# Autodesk Inventor assembly: Assembly1
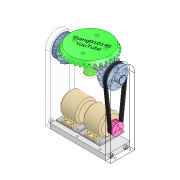
[picture p0: Inventor's stored thumbnail of the model, 180x180]
Saved by Autodesk Inventor 2022.5 (Build 265521000, 521)
## iProperties
Created: 2020-07-24
Part Number: Assembly1
Document SubType Name: Assembly
Designer: admin
Author: admin
## Documents named in this file (12)
- F:\YouTube\2024\YouTube\11N\6BevelGear2DoF\Assembly0.iam
- F:\YouTube\2024\YouTube\11N\6BevelGear2DoF\B32x2i2.ipt
- F:\YouTube\2024\YouTube\11N\6BevelGear2DoF\B16x2i2.ipt
- F:\YouTube\2024\YouTube\11N\6BevelGear2DoF\Cross.ipt
- F:\YouTube\2024\YouTube\11N\6BevelGear2DoF\Bearing.ipt
- F:\YouTube\2024\YouTube\11N\6BevelGear2DoF\Bottom.ipt
- F:\YouTube\2024\YouTube\11N\6BevelGear2DoF\Motor1x40.ipt
- F:\YouTube\2024\YouTube\11N\6BevelGear2DoF\Pulley.ipt
- F:\YouTube\2024\YouTube\11N\6BevelGear2DoF\Belt.ipt
- F:\YouTube\2024\YouTube\11N\6BevelGear2DoF\MotorBase.ipt
- F:\YouTube\2024\YouTube\11N\6BevelGear2DoF\PinScrew.ipt
- F:\YouTube\2024\YouTube\11N\6BevelGear2DoF\Nut3.ipt
## Components (16 placed, 11 different names)
1. Motor1x40:1 — Mate:18, Mate:19, Flush:4, Mate:22, Mate:23, Mate:25, Mate:31, Flush:6
2. Motor1x40:2 — Mate:21, Flush:4, Mate:32
3. Bearing:1 — Mate:12, Mate:13, Angle:1, Flush:1, Mate:18, Mate:24, Mate:26, Mate:27, Mate:28
4. Bearing:2 — Mate:14, Mate:15, Flush:1, Flush:2, Flush:3, Mate:16, Mate:21, Mate:33
5. Bottom:1 — Flush:2, Flush:3, Mate:16, Flush:5
6. Belt:1 — Mate:24, Mate:25, Mate:26
7. MotorBase:1 — Mate:31, Flush:5, Flush:6, Flush:7
8. MotorBase:2 — Mate:32, Flush:7, Mate:33, Insert:1, Insert:2, Insert:3
9. PinScrew:1 — Insert:1
10. Nut3:1 — Insert:2
11. Nut3:2 — Insert:3
12. B32x2i2:1 — Mate:29, Mate:30, Angle:2
13. B16x2i2:1 — Mate:3, Mate:4, Mate:5, Mate:7, Mate:12, Mate:13
14. B16x2i2:2 — Mate:6, Mate:7, Mate:14, Mate:15
15. Cross:1 — Mate:27, Mate:28, Mate:29, Mate:30
16. Pulley:1 — Mate:22, Mate:23
## Relationships (37: Mate 25, Flush 7, Insert 3, Angle 2)
- Mate:3: B16x2i2:1
- Mate:4: B16x2i2:1
- Mate:5: B16x2i2:1
- Mate:6: B16x2i2:2
- Mate:7: B16x2i2:1 ↔ B16x2i2:2
- Mate:12: Bearing:1 ↔ B16x2i2:1
- Mate:13: Bearing:1 ↔ B16x2i2:1
- Angle:1 (0 deg): Bearing:1
- Mate:14: Bearing:2 ↔ B16x2i2:2
- Mate:15: Bearing:2 ↔ B16x2i2:2
- Flush:1: Bearing:1 ↔ Bearing:2
- Flush:2: Bearing:2 ↔ Bottom:1
- Flush:3: Bearing:2 ↔ Bottom:1
- Mate:16: Bearing:2 ↔ Bottom:1
- Mate:18 (12 mm): Motor1x40:1 ↔ Bearing:1
- Mate:19: Motor1x40:1
- Mate:21 (12 mm): Motor1x40:2 ↔ Bearing:2
- Flush:4: Motor1x40:1 ↔ Motor1x40:2
- Mate:22 (4 mm): Motor1x40:1 ↔ Pulley:1
- Mate:23: Motor1x40:1 ↔ Pulley:1
- Mate:24: Bearing:1 ↔ Belt:1
- Mate:25: Motor1x40:1 ↔ Belt:1
- Mate:26 (1 mm): Bearing:1 ↔ Belt:1
- Mate:27: Bearing:1 ↔ Cross:1
- Mate:28 (20 mm): Bearing:1 ↔ Cross:1
- Mate:29: B32x2i2:1 ↔ Cross:1
- Mate:30: B32x2i2:1 ↔ Cross:1
- Mate:31: Motor1x40:1 ↔ MotorBase:1
- Flush:5: Bottom:1 ↔ MotorBase:1
- Flush:6 (2.5 mm): Motor1x40:1 ↔ MotorBase:1
- Mate:32: Motor1x40:2 ↔ MotorBase:2
- Flush:7: MotorBase:1 ↔ MotorBase:2
- Mate:33 (10 mm): Bearing:2 ↔ MotorBase:2
- Insert:1 (3 mm): MotorBase:2 ↔ PinScrew:1
- Insert:2: MotorBase:2 ↔ Nut3:1
- Insert:3: MotorBase:2 ↔ Nut3:2
- Angle:2 (0 deg): B32x2i2:1
